# Autodesk Inventor assembly: WalkerAssembly
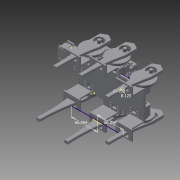
[picture p0: Inventor's stored thumbnail of the model, 180x180]
Saved by Autodesk Inventor 2015 (Build 190159000, 159)
## iProperties
Created: 2016-04-26
Part Number: WalkerAssembly
Document SubType Name: Assembly
Designer: Hatch
Author: Hatch
## Documents named in this file (8)
- C:\Users\Hatch\Documents\WalkerAssembly.iam
- C:\Users\Hatch\Documents\WalkerBase.ipt
- C:\Users\Hatch\Documents\LegWheel.ipt
- C:\Users\Hatch\Documents\Leg.ipt
- C:\Users\Hatch\Documents\XL-320(stp)\Imported Components\XL-320\XL-320.ipt
- C:\Users\Hatch\Documents\RPiCaseV2.ipt
- C:\Users\Hatch\Documents\RPiCaseTop.ipt
- C:\Users\Hatch\Documents\ClawJoint.ipt
## Components (24 placed, 7 different names)
1. WalkerBase:1 — Insert:2, Insert:3, Insert:6, Insert:7, Insert:12, Insert:13, Insert:15, Insert:16, Insert:17, Insert:20, Insert:21, Insert:28
2. LegWheel:1 — Insert:1, Mate:1, Insert:25
3. LegWheel:2 — Insert:19, Mate:2, Insert:26
4. LegWheel:3 — Insert:18, Mate:3, Insert:27
5. Leg:1 — Mate:2, Insert:26
6. Leg:2 — Mate:3, Insert:27
7. Leg:3 — Mate:1, Insert:25
8. XL-320:1 — Insert:31, Insert:32
9. XL-320:2 — Insert:1, Insert:2, Insert:3, Insert:33
10. XL-320:3 — Insert:4, Insert:5, Insert:6, Insert:7, Mate:7
11. XL-320:4 — Insert:10, Insert:11, Insert:20, Insert:21
12. XL-320:5 — Insert:12, Insert:13, Insert:14
13. XL-320:6 — Insert:15, Insert:29, Insert:30
14. XL-320:7 — Insert:16, Insert:19, Insert:28
15. XL-320:8 — Insert:17, Insert:18
16. LegWheel:4 — Insert:4, Insert:5, Mate:6, Insert:23
17. LegWheel:5 — Insert:14, Mate:4, Insert:24
18. LegWheel:6 — Insert:10, Insert:11, Insert:22
19. Leg:4 — Mate:6, Insert:23
20. Leg:5 — Insert:22
21. Leg:6 — Mate:4, Insert:24
22. RPiCaseV2:1 — Mate:7, Insert:33, Insert:34
23. RPiCaseTop:1 — Insert:34
24. ClawJoint:1 — Insert:29, Insert:30, Insert:31, Insert:32
## Relationships (38: Insert 32, Mate 6)
- Insert:1: LegWheel:1 ↔ XL-320:2
- Insert:2: WalkerBase:1 ↔ XL-320:2
- Insert:3: WalkerBase:1 ↔ XL-320:2
- Mate:1: LegWheel:1 ↔ Leg:3
- Insert:4: XL-320:3 ↔ LegWheel:4
- Insert:5: XL-320:3 ↔ LegWheel:4
- Insert:6: WalkerBase:1 ↔ XL-320:3
- Insert:7: WalkerBase:1 ↔ XL-320:3
- Insert:10: XL-320:4 ↔ LegWheel:6
- Insert:11: XL-320:4 ↔ LegWheel:6
- Insert:12: WalkerBase:1 ↔ XL-320:5
- Insert:13: WalkerBase:1 ↔ XL-320:5
- Insert:14: XL-320:5 ↔ LegWheel:5
- Insert:15: WalkerBase:1 ↔ XL-320:6
- Insert:16: WalkerBase:1 ↔ XL-320:7
- Insert:17: WalkerBase:1 ↔ XL-320:8
- Insert:18: LegWheel:3 ↔ XL-320:8
- Insert:19: LegWheel:2 ↔ XL-320:7
- Mate:2: LegWheel:2 ↔ Leg:1
- Mate:3: LegWheel:3 ↔ Leg:2
- Mate:4: LegWheel:5 ↔ Leg:6
- Mate:6: LegWheel:4 ↔ Leg:4
- Insert:20: WalkerBase:1 ↔ XL-320:4
- Insert:21: WalkerBase:1 ↔ XL-320:4
- Insert:22: LegWheel:6 ↔ Leg:5
- Insert:23: LegWheel:4 ↔ Leg:4
- Insert:24: LegWheel:5 ↔ Leg:6
- Insert:25: LegWheel:1 ↔ Leg:3
- Insert:26: LegWheel:2 ↔ Leg:1
- Insert:27: LegWheel:3 ↔ Leg:2
- Insert:28: WalkerBase:1 ↔ XL-320:7
- Insert:29: XL-320:6 ↔ ClawJoint:1
- Insert:30: XL-320:6 ↔ ClawJoint:1
- Insert:31: XL-320:1 ↔ ClawJoint:1
- Insert:32: XL-320:1 ↔ ClawJoint:1
- Mate:7: XL-320:3 ↔ RPiCaseV2:1
- Insert:33: XL-320:2 ↔ RPiCaseV2:1
- Insert:34: RPiCaseV2:1 ↔ RPiCaseTop:1
